# Autodesk Inventor assembly: SeatAssembly
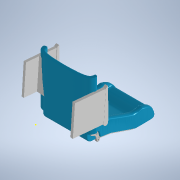
[picture p0: Inventor's stored thumbnail of the model, 180x180]
Saved by Autodesk Inventor 2021 (Build 250183000, 183)
## iProperties
Created: 2021-01-30
Part Number: SeatAssembly
Document SubType Name: Assembly
Designer: argon
Author: argon
## Documents named in this file (7)
- C:\Users\ahuja\Documents\GrabCAD\EngOne Maroons - MDL CAD Designathon 2021\Arm Rest\SeatAssembly.iam
- C:\Users\ahuja\Documents\GrabCAD\EngOne Maroons - MDL CAD Designathon 2021\Arm Rest\SeatBack.ipt
- C:\Users\ahuja\Documents\GrabCAD\EngOne Maroons - MDL CAD Designathon 2021\Arm Rest\SteelPost.ipt
- C:\Users\ahuja\Documents\GrabCAD\EngOne Maroons - MDL CAD Designathon 2021\Arm Rest\SteelBack.ipt
- C:\Users\ahuja\Documents\GrabCAD\EngOne Maroons - MDL CAD Designathon 2021\Arm Rest\SeatBase.ipt
- C:\Users\ahuja\Documents\GrabCAD\EngOne Maroons - MDL CAD Designathon 2021\Arm Rest\handle 1.ipt
- C:\Users\ahuja\Documents\GrabCAD\EngOne Maroons - MDL CAD Designathon 2021\Arm Rest\handle 2.ipt
## Components (7 placed, 6 different names)
1. SeatBack:1 — Mate:1, Mate:2, Mate:3, Mate:4, Mate:7, Mate:8, Mate:9
2. SteelPost:1 — Mate:1, Mate:4, Mate:5
3. SteelPost:2 — Mate:2, Mate:3, Mate:5
4. SteelBack:1 — Mate:7, Mate:8, Mate:9
5. SeatBase:1
6. handle 1:1
7. handle 2:1
## Relationships (8: Mate 8)
- Mate:1: SeatBack:1 ↔ SteelPost:1
- Mate:2: SeatBack:1 ↔ SteelPost:2
- Mate:3: SeatBack:1 ↔ SteelPost:2
- Mate:4: SeatBack:1 ↔ SteelPost:1
- Mate:5: SteelPost:1 ↔ SteelPost:2
- Mate:7: SeatBack:1 ↔ SteelBack:1
- Mate:8: SeatBack:1 ↔ SteelBack:1
- Mate:9: SeatBack:1 ↔ SteelBack:1
